# Autodesk Inventor assembly: EnsambleMecanismoEnsayo
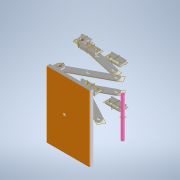
[picture p0: Inventor's stored thumbnail of the model, 180x180]
Saved by Autodesk Inventor 2021 (Build 250183000, 183)
## iProperties
Created: 2021-04-17
Part Number: EnsambleMecanismoEnsayo
Document SubType Name: Assembly
Designer: GABRIEL LOL
Author: GABRIEL LOL
## Documents named in this file (9)
- J:\PAI\Proyecto_PAI_2021\01 CAD\EnsambleMecanismoEnsayo.iam
- J:\PAI\Proyecto_PAI_2021\01 CAD\PasadorPivotePreliminar.ipt
- J:\PAI\Proyecto_PAI_2021\01 CAD\EslabonPreliminarElevacion.ipt
- J:\PAI\Proyecto_PAI_2021\01 CAD\ApoyoRotatorioPreliminar.ipt
- J:\PAI\Proyecto_PAI_2021\01 CAD\PistaEslabonPreliminar.ipt
- J:\PAI\Proyecto_PAI_2021\01 CAD\SoporteBaseElevacion.ipt
- J:\PAI\Proyecto_PAI_2021\01 CAD\BaseExtrusion.ipt
- J:\PAI\Proyecto_PAI_2021\01 CAD\PisoDeEnsayoIgnorar.ipt
- C:\Users\GABRIEL LOL\OneDrive - Universidad Nacional de Colombia\PAI\3_Producto 3D\PasadorPreliminar.ipt
## Components (20 placed, 8 different names)
1. PasadorPivotePreliminar:1 — Mate:31, Flush:16, Mate:32
2. EslabonPreliminarElevacion:1 — Mate:29, Flush:15, Flush:24
3. ApoyoRotatorioPreliminar:1 — Mate:32, Flush:17, Mate:33, Flush:21
4. EslabonPreliminarElevacion:2 — Mate:3, Mate:4, Mate:6
5. EslabonPreliminarElevacion:3 — Mate:31, Flush:16, Flush:17
6. EslabonPreliminarElevacion:4 — Mate:14, Mate:15, Flush:7
7. ApoyoRotatorioPreliminar:2 — Mate:30, Flush:14, Flush:15, Mate:34, Flush:20
8. ApoyoRotatorioPreliminar:3 — Mate:2, Mate:7, Flush:3, Mate:14, Mate:16
9. ApoyoRotatorioPreliminar:4 — Mate:1, Mate:5, Mate:6, Mate:7, Flush:2, Flush:3, Flush:4, Mate:21, Mate:22
10. PasadorPivotePreliminar:2 — Mate:29, Mate:30, Flush:14
11. PasadorPivotePreliminar:3 — Mate:15, Flush:7, Mate:16
12. PasadorPivotePreliminar:4 — Mate:3, Mate:4, Mate:5
13. PistaEslabonPreliminar:1 — Mate:20, Mate:23, Mate:24
14. PistaEslabonPreliminar:2 — Mate:19, Mate:21, Mate:22, Mate:23, Mate:24, Flush:25
15. SoporteBaseElevacion:1 — Mate:8, Mate:9, Mate:10, Mate:33, Mate:34, Mate:35, Mate:36, Flush:20, Flush:21
16. BaseExtrusion:1 — Mate:8, Mate:9, Mate:10
17. PisoDeEnsayoIgnorar:1 — Mate:1, Mate:2, Flush:2, Flush:4, Mate:19, Mate:20
18. PistaEslabonPreliminar:3 — Mate:35, Flush:22, Flush:23, Flush:25
19. PistaEslabonPreliminar:4 — Mate:36, Flush:22, Flush:23, Flush:24
20. PasadorPreliminar:1
## Relationships (41: Mate 27, Flush 14)
- Mate:1: ApoyoRotatorioPreliminar:4 ↔ PisoDeEnsayoIgnorar:1
- Mate:2: ApoyoRotatorioPreliminar:3 ↔ PisoDeEnsayoIgnorar:1
- Mate:3: EslabonPreliminarElevacion:2 ↔ PasadorPivotePreliminar:4
- Mate:4: EslabonPreliminarElevacion:2 ↔ PasadorPivotePreliminar:4
- Mate:5: ApoyoRotatorioPreliminar:4 ↔ PasadorPivotePreliminar:4
- Mate:6: EslabonPreliminarElevacion:2 ↔ ApoyoRotatorioPreliminar:4
- Mate:7: ApoyoRotatorioPreliminar:3 ↔ ApoyoRotatorioPreliminar:4
- Mate:8: SoporteBaseElevacion:1 ↔ BaseExtrusion:1
- Mate:9: SoporteBaseElevacion:1 ↔ BaseExtrusion:1
- Mate:10: SoporteBaseElevacion:1 ↔ BaseExtrusion:1
- Flush:2: ApoyoRotatorioPreliminar:4 ↔ PisoDeEnsayoIgnorar:1
- Flush:3 (250 mm): ApoyoRotatorioPreliminar:3 ↔ ApoyoRotatorioPreliminar:4
- Flush:4 (108 mm): ApoyoRotatorioPreliminar:4 ↔ PisoDeEnsayoIgnorar:1
- Mate:14: EslabonPreliminarElevacion:4 ↔ ApoyoRotatorioPreliminar:3
- Mate:15: EslabonPreliminarElevacion:4 ↔ PasadorPivotePreliminar:3
- Flush:7: EslabonPreliminarElevacion:4 ↔ PasadorPivotePreliminar:3
- Mate:16: ApoyoRotatorioPreliminar:3 ↔ PasadorPivotePreliminar:3
- Mate:19: PistaEslabonPreliminar:2 ↔ PisoDeEnsayoIgnorar:1
- Mate:20: PistaEslabonPreliminar:1 ↔ PisoDeEnsayoIgnorar:1
- Mate:21: ApoyoRotatorioPreliminar:4 ↔ PistaEslabonPreliminar:2
- Mate:22 (173.4 mm): ApoyoRotatorioPreliminar:4 ↔ PistaEslabonPreliminar:2
- Mate:23: PistaEslabonPreliminar:1 ↔ PistaEslabonPreliminar:2
- Mate:24 (-250 mm): PistaEslabonPreliminar:1 ↔ PistaEslabonPreliminar:2
- Mate:29: EslabonPreliminarElevacion:1 ↔ PasadorPivotePreliminar:2
- Mate:30: ApoyoRotatorioPreliminar:2 ↔ PasadorPivotePreliminar:2
- Flush:14: ApoyoRotatorioPreliminar:2 ↔ PasadorPivotePreliminar:2
- Flush:15: EslabonPreliminarElevacion:1 ↔ ApoyoRotatorioPreliminar:2
- Mate:31: PasadorPivotePreliminar:1 ↔ EslabonPreliminarElevacion:3
- Flush:16: PasadorPivotePreliminar:1 ↔ EslabonPreliminarElevacion:3
- Mate:32: PasadorPivotePreliminar:1 ↔ ApoyoRotatorioPreliminar:1
- Flush:17: ApoyoRotatorioPreliminar:1 ↔ EslabonPreliminarElevacion:3
- Mate:33: ApoyoRotatorioPreliminar:1 ↔ SoporteBaseElevacion:1
- Mate:34: ApoyoRotatorioPreliminar:2 ↔ SoporteBaseElevacion:1
- Mate:35: SoporteBaseElevacion:1 ↔ PistaEslabonPreliminar:3
- Mate:36: SoporteBaseElevacion:1 ↔ PistaEslabonPreliminar:4
- Flush:20: ApoyoRotatorioPreliminar:2 ↔ SoporteBaseElevacion:1
- Flush:21 (-105 mm): ApoyoRotatorioPreliminar:1 ↔ SoporteBaseElevacion:1
- Flush:22: PistaEslabonPreliminar:3 ↔ PistaEslabonPreliminar:4
- Flush:23 (220 mm): PistaEslabonPreliminar:3 ↔ PistaEslabonPreliminar:4
- Flush:24: EslabonPreliminarElevacion:1 ↔ PistaEslabonPreliminar:4
- Flush:25: PistaEslabonPreliminar:2 ↔ PistaEslabonPreliminar:3
